# Autodesk Inventor assembly: Hub
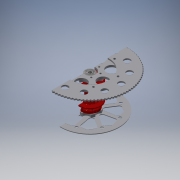
[picture p0: Inventor's stored thumbnail of the model, 180x180]
Saved by Autodesk Inventor 2018 (Build 220112000, 112)
## iProperties
Created: 2018-01-25
Part Number: Hub
Document SubType Name: Assembly
Designer: eroldan
Author: eroldan
## Documents named in this file (9)
- C:\Users\eroldan\Desktop\3dprojects\OpenEmoto\Hub\Hub.iam
- C:\Users\eroldan\Desktop\3dprojects\OpenEmoto\Hub\Hub.ipt
- C:\Users\eroldan\Desktop\3dprojects\OpenEmoto\Hub\ScrewAdapterPlate.ipt
- C:\Users\eroldan\Desktop\3dprojects\OpenEmoto\Hub\SprocketHubPlate.ipt
- C:\Users\eroldan\Desktop\3dprojects\OpenEmoto\OtherParts\Sprocket92T.ipt
- C:\Users\eroldan\Desktop\3dprojects\OpenEmoto\Hub\Spacer8mm.ipt
- C:\Users\eroldan\Desktop\3dprojects\OpenEmoto\OtherParts\DiskBrake180.ipt
- C:\Users\eroldan\Desktop\3dprojects\OpenEmoto\Hub\BearingsSpacer.ipt
- C:\Users\eroldan\Desktop\3dprojects\OpenEmoto\Hub\DesignAccelerator\Bearing1.iam
## Components (9 placed, 8 different names)
1. Sprocket92T:1
2. ScrewAdapterPlate:1 — Mate:14, Mate:15
3. SprocketHubPlate:1 — Mate:14, Mate:15
4. Hub:1 — Insert:1, Insert:2
5. Spacer8mm:1
6. DiskBrake180:1
7. BearingsSpacer:1 — Flush:1
8. Bearing:1 [sub-assembly] — Insert:1
9. Bearing:2 [sub-assembly] — Insert:2
## Relationships (16: Mate 13, Insert 2, Flush 1)
- [Mate]: ScrewAdapterPlate:1 ↔ Hub:1
- [Mate]: Sprocket92T:1 ↔ Hub:1
- [Mate]: Sprocket92T:1 ↔ SprocketHubPlate:1
- [Mate]: Sprocket92T:1 ↔ SprocketHubPlate:1
- [Mate]: Sprocket92T:1 ↔ SprocketHubPlate:1
- [Mate]: Hub:1 ↔ Spacer8mm:1
- [Mate]: Hub:1 ↔ Spacer8mm:1
- [Mate]: Hub:1 ↔ Spacer8mm:1
- [Mate]: Spacer8mm:1 ↔ DiskBrake180:1
- [Mate]: Spacer8mm:1 ↔ DiskBrake180:1
- [Mate]: Spacer8mm:1 ↔ DiskBrake180:1
- Flush:1: BearingsSpacer:1
- Insert:1: Hub:1 ↔ Bearing:1
- Insert:2: Hub:1 ↔ Bearing:2
- Mate:14: ScrewAdapterPlate:1 ↔ SprocketHubPlate:1
- Mate:15: ScrewAdapterPlate:1 ↔ SprocketHubPlate:1
